# Autodesk Inventor assembly: CP1x1 test assembly
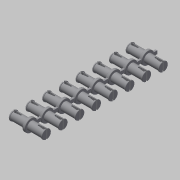
[picture p0: Inventor's stored thumbnail of the model, 180x180]
Saved by Autodesk Inventor 2019.3 (Build 233278000, 278)
## iProperties
Created: 2019-02-28
Part Number: CP1x1 test assembly
Document SubType Name: Assembly
Designer: Varga Daniel
Author: Varga Daniel
## Documents named in this file (11)
- C:\!_Dani\!_cloud\OneDrive\!_munka\Revolution\RevvyDemoKit\Structural parts\RFQ\SLS print collection Rev 1\CP1x1\CP1x1 test assembly.iam
- C:\!_Dani\!_cloud\OneDrive\!_munka\Revolution\RevvyDemoKit\Structural parts\RFQ\SLS print collection Rev 1\CP1x1\CP1x1_4,850_8,500.ipt
- C:\!_Dani\!_cloud\OneDrive\!_munka\Revolution\RevvyDemoKit\Structural parts\RFQ\SLS print collection Rev 1\CP1x1.ipt
- C:\!_Dani\!_cloud\OneDrive\!_munka\Revolution\RevvyDemoKit\Structural parts\RFQ\SLS print collection Rev 1\CP1x1\CP1x1_4,875_8,500.ipt
- C:\!_Dani\!_cloud\OneDrive\!_munka\Revolution\RevvyDemoKit\Structural parts\RFQ\SLS print collection Rev 1\CP1x1\CP1x1_4,900_8,400.ipt
- C:\!_Dani\!_cloud\OneDrive\!_munka\Revolution\RevvyDemoKit\Structural parts\RFQ\SLS print collection Rev 1\CP1x1\CP1x1_4,900_8,425.ipt
- C:\!_Dani\!_cloud\OneDrive\!_munka\Revolution\RevvyDemoKit\Structural parts\RFQ\SLS print collection Rev 1\CP1x1\CP1x1_4,900_8,450.ipt
- C:\!_Dani\!_cloud\OneDrive\!_munka\Revolution\RevvyDemoKit\Structural parts\RFQ\SLS print collection Rev 1\CP1x1\CP1x1_4,900_8,500.ipt
- C:\!_Dani\!_cloud\OneDrive\!_munka\Revolution\RevvyDemoKit\Structural parts\RFQ\SLS print collection Rev 1\CP1x1\CP1x1_4,925_8,500.ipt
- C:\!_Dani\!_cloud\OneDrive\!_munka\Revolution\RevvyDemoKit\Structural parts\RFQ\SLS print collection Rev 1\CP1x1\CP1x1_4,950_8,500.ipt
- C:\!_Dani\!_cloud\OneDrive\!_munka\Revolution\RevvyDemoKit\Structural parts\RFQ\SLS print collection Rev 1\CP1x1\pin_interconnect.ipt
## Components (9 placed, 9 different names)
1. CP1x1_4,950_8,500:8 — Tangent:1, Flush:1, Flush:2, Flush:3, Flush:4, Flush:5, Flush:6, Flush:7, Flush:8, Mate:1, Flush:9
2. CP1x1_4,925_8,500:7 — Tangent:2, Flush:1, Flush:9, Flush:10
3. CP1x1_4,900_8,500:6 — Tangent:3, Flush:2, Flush:10, Flush:11
4. CP1x1_4,875_8,500:2 — Tangent:4, Flush:3, Flush:11, Flush:12
5. CP1x1_4,850_8,500:1 — Tangent:5, Flush:4, Flush:12, Flush:13
6. CP1x1_4,900_8,400:3 — Tangent:6, Flush:5, Flush:13, Flush:14
7. CP1x1_4,900_8,425:4 — Tangent:7, Flush:6, Flush:14, Flush:15
8. CP1x1_4,900_8,450:5 — Tangent:8, Flush:7, Flush:15
9. pin_interconnect:2 — Flush:8, Mate:1, Angle:1
## Relationships (25: Flush 15, Tangent 8, Mate 1, Angle 1)
- Tangent:1: CP1x1_4,950_8,500:8
- Tangent:2: CP1x1_4,925_8,500:7
- Tangent:3: CP1x1_4,900_8,500:6
- Tangent:4: CP1x1_4,875_8,500:2
- Tangent:5: CP1x1_4,850_8,500:1
- Tangent:6: CP1x1_4,900_8,400:3
- Tangent:7: CP1x1_4,900_8,425:4
- Tangent:8: CP1x1_4,900_8,450:5
- Flush:1: CP1x1_4,950_8,500:8 ↔ CP1x1_4,925_8,500:7
- Flush:2: CP1x1_4,950_8,500:8 ↔ CP1x1_4,900_8,500:6
- Flush:3: CP1x1_4,950_8,500:8 ↔ CP1x1_4,875_8,500:2
- Flush:4: CP1x1_4,950_8,500:8 ↔ CP1x1_4,850_8,500:1
- Flush:5: CP1x1_4,950_8,500:8 ↔ CP1x1_4,900_8,400:3
- Flush:6: CP1x1_4,950_8,500:8 ↔ CP1x1_4,900_8,425:4
- Flush:7: CP1x1_4,950_8,500:8 ↔ CP1x1_4,900_8,450:5
- Flush:8 (0.3 mm): CP1x1_4,950_8,500:8 ↔ pin_interconnect:2
- Mate:1: CP1x1_4,950_8,500:8 ↔ pin_interconnect:2
- Flush:9 (10 mm): CP1x1_4,950_8,500:8 ↔ CP1x1_4,925_8,500:7
- Flush:10 (10 mm): CP1x1_4,925_8,500:7 ↔ CP1x1_4,900_8,500:6
- Flush:11 (10 mm): CP1x1_4,900_8,500:6 ↔ CP1x1_4,875_8,500:2
- Flush:12 (10 mm): CP1x1_4,875_8,500:2 ↔ CP1x1_4,850_8,500:1
- Flush:13 (10 mm): CP1x1_4,850_8,500:1 ↔ CP1x1_4,900_8,400:3
- Flush:14 (10 mm): CP1x1_4,900_8,400:3 ↔ CP1x1_4,900_8,425:4
- Flush:15 (10 mm): CP1x1_4,900_8,425:4 ↔ CP1x1_4,900_8,450:5
- Angle:1 (180 deg): pin_interconnect:2
